# Autodesk Inventor assembly: Arm2
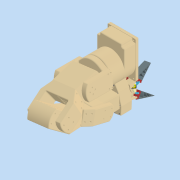
[picture p0: Inventor's stored thumbnail of the model, 180x180]
Saved by Autodesk Inventor 2020.2 (Build 242310000, 310)
## iProperties
Created: 2020-02-07
Part Number: Arm2
Document SubType Name: Assembly
Designer: JochenAlt
Author: JochenAlt
## Documents named in this file (9)
- D:\Projects\MiniBot\CAD\Arm.iam
- D:\Projects\MiniBot\CAD\Elbow.iam
- D:\Projects\MiniBot\CAD\Upperarm.iam
- D:\Projects\MiniBot\CAD\Base.iam
- D:\Projects\MiniBot\CAD\Forearm.iam
- D:\Projects\MiniBot\CAD\Shoulder.iam
- D:\Projects\MiniBot\CAD\Wrist.iam
- D:\Projects\MiniBot\CAD\gripper\Gripper.iam
- D:\Projects\MiniBot\CAD\extern\electronics\Odroid C2\ODroid C2.iam
## Components (8 placed, 8 different names)
1. Upperarm:1 [sub-assembly] — Passend:69, Passend:70, Passend:82, Passend:83
2. Base:1 [sub-assembly] — Passend:61, Fluchtend:1, Fluchtend:2
3. Shoulder:1 [sub-assembly] — Passend:61, Fluchtend:1, Passend:82, Passend:83
4. Elbow:2 [sub-assembly] — Passend:69, Passend:70, Passend:77, Passend:78
5. Wrist:3 [sub-assembly] — Passend:75, Passend:79, Passend:80, Passend:81, Passend:84
6. Gripper:1 [sub-assembly] — Passend:75, Passend:81, Passend:84
7. Forearm:1 [sub-assembly] — Passend:77, Passend:78, Passend:79, Passend:80
8. ODroid C2:1 [sub-assembly] — Fluchtend:2
## Relationships (14: Mate 12, Flush 2)
- Passend:61 [Mate]: Base:1 ↔ Shoulder:1
- Fluchtend:1 [Flush]: Base:1 ↔ Shoulder:1
- Passend:69 [Mate]: Upperarm:1 ↔ Elbow:2
- Passend:70 [Mate]: Upperarm:1 ↔ Elbow:2
- Passend:75 [Mate]: Wrist:3 ↔ Gripper:1
- Passend:77 [Mate]: Elbow:2 ↔ Forearm:1
- Passend:78 [Mate]: Elbow:2 ↔ Forearm:1
- Passend:79 [Mate]: Wrist:3 ↔ Forearm:1
- Passend:80 [Mate]: Wrist:3 ↔ Forearm:1
- Passend:81 [Mate]: Wrist:3 ↔ Gripper:1
- Fluchtend:2 [Flush]: Base:1 ↔ ODroid C2:1
- Passend:82 [Mate]: Upperarm:1 ↔ Shoulder:1
- Passend:83 [Mate]: Upperarm:1 ↔ Shoulder:1
- Passend:84 [Mate]: Wrist:3 ↔ Gripper:1
